# Autodesk Inventor assembly: mechanum wheel
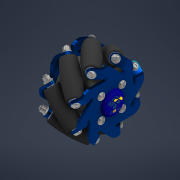
[picture p0: Inventor's stored thumbnail of the model, 180x180]
Saved by Autodesk Inventor 2021.3 (Build 253353000, 353)
## iProperties
Created: 2021-10-17
Part Number: mechanum wheel
Document SubType Name: Assembly
Designer: ASUS
Author: ASUS
## Documents named in this file (9)
- E:\Inventor\mecanum wheel\mechanum wheel.iam
- E:\Inventor\mecanum wheel\shaft.ipt
- E:\Inventor\mecanum wheel\frame.ipt
- E:\Inventor\mecanum wheel\bolt.ipt
- C:\Users\ASUS\Documents\Inventor\Content Center Files\R2021\en-US\ISO 10511\ISO 10511 - M3.ipt
- E:\Inventor\mecanum wheel\roller.ipt
- E:\Inventor\mecanum wheel\roller bracket.ipt
- E:\Inventor\mecanum wheel\roller bracket_MIR.ipt
- E:\Inventor\mecanum wheel\tutup.ipt
## Components (53 placed, 8 different names)
1. shaft:1 — Mate:1, Mate:2, Mate:3, Mate:4, Mate:5, Mate:6, Mate:7, Mate:8, Mate:21
2. frame:1 — Mate:4, Mate:5, Mate:6, Rotational:1, Mate:15, Mate:18
3. frame:2 — Mate:7, Mate:8, Rigid:1, Mate:13, Mate:14, Mate:17, Mate:22
4. roller:5
5. tutup:1 — Mate:21, Mate:22
6. bolt:1 — Rigid:1
7. bolt:2
8. bolt:3
9. bolt:4
10. DIN EN ISO 10511 M3:2 — Rotational:1
11. DIN EN ISO 10511 M3:3
12. DIN EN ISO 10511 M3:4
13. DIN EN ISO 10511 M3:5
14. bolt:5 — Mate:16, Mate:17, Mate:19, Mate:20
15. roller:1 — Mate:9, Mate:10, Mate:11, Mate:12, Mate:14, Mate:15, Mate:16
16. roller bracket:1 — Mate:9, Mate:10, Mate:13
17. roller bracket_MIR:1 — Mate:11, Mate:12
18. DIN EN ISO 10511 M3:6 — Mate:18, Mate:19, Mate:20
19. bolt:6
20. roller:2
21. roller bracket:2
22. roller bracket_MIR:2
23. DIN EN ISO 10511 M3:7
24. bolt:7
25. roller:3
26. roller bracket:3
27. roller bracket_MIR:3
28. DIN EN ISO 10511 M3:8
29. bolt:8
30. roller:4
31. roller bracket:4
32. roller bracket_MIR:4
33. DIN EN ISO 10511 M3:9
34. bolt:10
35. roller:6
36. roller bracket:8
37. roller bracket_MIR:5
38. DIN EN ISO 10511 M3:10
39. bolt:11
40. roller:7
41. roller bracket:9
42. roller bracket_MIR:6
43. DIN EN ISO 10511 M3:11
44. bolt:12
45. roller:8
46. roller bracket:10
47. roller bracket_MIR:7
48. DIN EN ISO 10511 M3:12
49. bolt:13
50. roller:9
51. roller bracket:11
52. roller bracket_MIR:8
53. DIN EN ISO 10511 M3:13
## Component patterns: (4 elements, first: bolt:1), (4 elements, first: DIN EN ISO 10511 M3:2), (8 elements, first: bolt:5 + roller:1 + roller bracket:1 + roller bracket_MIR:1 + DIN EN ISO 10511 M3:6)
## Relationships (24: Mate 22, WeldJoint 1, RevoluteJoint 1)
- Mate:1: shaft:1
- Mate:2: shaft:1
- Mate:3: shaft:1
- Mate:4: shaft:1 ↔ frame:1
- Mate:5: shaft:1 ↔ frame:1
- Mate:6: shaft:1 ↔ frame:1
- Mate:7: shaft:1 ↔ frame:2
- Mate:8: shaft:1 ↔ frame:2
- Rigid:1 [WeldJoint]: frame:2 ↔ bolt:1
- Rotational:1 [RevoluteJoint]: frame:1 ↔ DIN EN ISO 10511 M3:2
- Mate:9: roller:1 ↔ roller bracket:1
- Mate:10: roller:1 ↔ roller bracket:1
- Mate:11: roller:1 ↔ roller bracket_MIR:1
- Mate:12: roller:1 ↔ roller bracket_MIR:1
- Mate:13: frame:2 ↔ roller bracket:1
- Mate:14: frame:2 ↔ roller:1
- Mate:15: frame:1 ↔ roller:1
- Mate:16: bolt:5 ↔ roller:1
- Mate:17: frame:2 ↔ bolt:5
- Mate:18: frame:1 ↔ DIN EN ISO 10511 M3:6
- Mate:19: bolt:5 ↔ DIN EN ISO 10511 M3:6
- Mate:20: bolt:5 ↔ DIN EN ISO 10511 M3:6
- Mate:21: shaft:1 ↔ tutup:1
- Mate:22: frame:2 ↔ tutup:1
